# Autodesk Inventor assembly: Assembly
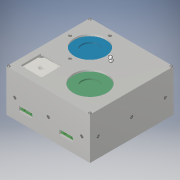
[picture p0: Inventor's stored thumbnail of the model, 180x180]
Saved by Autodesk Inventor 2018 (Build 220112000, 112)
## iProperties
Created: 2021-04-18
Part Number: Assembly
Document SubType Name: Assembly
Designer: Ramana Bharathi
Mass: 2974.86 g
Surface Area: 6185.71 cm^2
Volume: 1496.71 cm^3
Density: 1.9876 g/cm^3
Author: Ramana Bharathi
## Documents named in this file (17)
- E:\College\college material\4th sem\Machining and precision manufacturing\Assignments\task-1\Assembly.iam
- E:\College\college material\4th sem\Machining and precision manufacturing\Assignments\task-1\sensor3.ipt
- E:\College\college material\4th sem\Machining and precision manufacturing\Assignments\task-1\sensor1.ipt
- E:\College\college material\4th sem\Machining and precision manufacturing\Assignments\task-1\sensor2.ipt
- E:\College\college material\4th sem\Machining and precision manufacturing\Assignments\task-1\Housing_bottom.ipt
- E:\College\college material\4th sem\Machining and precision manufacturing\Assignments\task-1\spacer.ipt
- E:\College\college material\4th sem\Machining and precision manufacturing\Assignments\task-1\Board.ipt
- E:\College\college material\4th sem\Machining and precision manufacturing\Assignments\task-1\Housing_top.ipt
- E:\College\college material\4th sem\Machining and precision manufacturing\Assignments\task-1\Housing_lid.ipt
- E:\College\college material\4th sem\Machining and precision manufacturing\Assignments\task-1\sensor1_lock.ipt
- E:\College\college material\4th sem\Machining and precision manufacturing\Assignments\task-1\sensor3_lock.ipt
- E:\College\college material\4th sem\Machining and precision manufacturing\Assignments\task-1\sensor2_lock.ipt
- C:\Users\Ramana Bharathi\Documents\Inventor\Content Center Files\R2018\en-US\AS 1427(05)\AS 1427 - M3 x 8(5) II.ipt
- C:\Users\Ramana Bharathi\Documents\Inventor\Content Center Files\R2018\en-US\AS 1427(05)\AS 1427 - M4 x 6(5) II.ipt
- C:\Users\Ramana Bharathi\Documents\Inventor\Content Center Files\R2018\en-US\AS 1427(04)\AS 1427 - M3 x 16(5) I.ipt
- C:\Users\Ramana Bharathi\Documents\Inventor\Content Center Files\R2018\en-US\AS 1112 (2)\AS 1112 - M3  Type 5.ipt
- C:\Users\Ramana Bharathi\Documents\Inventor\Content Center Files\R2018\en-US\AS 1427(04)\AS 1427 - M4 x 8(5) I.ipt
## Components (63 placed, 16 different names)
1. sensor1:1 — Mate:2, Mate:3, Mate:5
2. sensor1:2 — Mate:4, Mate:5, Mate:7
3. sensor1:3 — Mate:6, Mate:7, Mate:8
4. sensor1:4 — Mate:1, Mate:8
5. sensor2:1 — Insert:16
6. sensor3:1 — Mate:46, Mate:47, Mate:48, Insert:12, Insert:13, Insert:14, Insert:15
7. Board:1 — Insert:17, Insert:18, Mate:63, Mate:65, Mate:67, Mate:69, Mate:71, Mate:73, Mate:77, Mate:79
8. Housing_bottom:1 — Insert:1, Insert:2, Insert:3, Insert:4, Insert:5, Insert:6, Insert:7, Insert:8, Insert:9, Flush:1, Flush:2, Mate:80, Mate:81, Mate:82, Mate:83, Mate:84, Mate:85, Mate:86, Mate:87, Mate:88, Mate:89, Mate:90, Mate:91, Mate:92
9. Housing_top:1 — Mate:40, Mate:41, Mate:42, Mate:43, Mate:44, Mate:45, Mate:53, Mate:54, Mate:55, Mate:60, Mate:61, Flush:1, Flush:2, Mate:80, Mate:93
10. Housing_lid:1 — Mate:9, Mate:10, Mate:11, Mate:12, Mate:36, Mate:37, Mate:38, Mate:39, Mate:60, Mate:61, Mate:93, Mate:94, Mate:95, Mate:96, Mate:97, Mate:98, Mate:99, Mate:100, Mate:101
11. spacer:1 — Insert:1, Insert:17, Mate:72
12. spacer:2 — Insert:2, Mate:68
13. spacer:3 — Insert:3, Mate:66
14. spacer:4 — Insert:4, Mate:76
15. spacer:5 — Insert:5
16. spacer:6 — Insert:6, Mate:64
17. spacer:7 — Insert:7, Mate:78
18. spacer:8 — Insert:8, Mate:70
19. spacer:9 — Insert:9, Insert:18, Mate:62
20. sensor1_lock:1 — Mate:1, Mate:2, Mate:3, Mate:4, Mate:6, Mate:9, Mate:10, Mate:11, Mate:12
21. AS 1427 H - Metric M4 x 8:11 — Mate:36
22. AS 1427 H - Metric M4 x 8:12 — Mate:37
23. AS 1427 H - Metric M4 x 8:13 — Mate:38
24. AS 1427 H - Metric M4 x 8:14 — Mate:39
25. sensor3_lock:1 — Mate:40, Mate:41, Mate:42, Mate:46, Mate:48, Insert:10, Insert:11
26. sensor3_lock:2 — Mate:43, Mate:44, Mate:45, Mate:47, Mate:49, Mate:50, Mate:51, Mate:52
27. sensor2_lock:1 — Mate:53, Mate:54, Insert:16, Mate:55, Mate:56, Mate:57, Mate:58, Mate:59
28. AS 1427 H - Metric M3 x 8:1 — Insert:10
29. AS 1427 H - Metric M3 x 8:2 — Insert:11
30. AS 1427 H - Metric M3 x 8:3 — Mate:49, Mate:50
31. AS 1427 H - Metric M3 x 8:4 — Mate:51, Mate:52
32. AS 1427 H - Metric M4 x 6:9 — Insert:12
33. AS 1427 H - Metric M4 x 6:10 — Insert:13
34. AS 1427 H - Metric M4 x 6:11 — Insert:14
35. AS 1427 H - Metric M4 x 6:12 — Insert:15
36. AS 1427 H - Metric M3 x 16:1 — Mate:56
37. AS 1427 H - Metric M3 x 16:2 — Mate:57
38. AS 1427 H - Metric M3 x 16:3 — Mate:58
39. AS 1427 H - Metric M3 x 16:4 — Mate:59
40. AS 1112 (2) - Metric M3  Type 5:1 — Mate:62, Mate:63
41. AS 1112 (2) - Metric M3  Type 5:2 — Mate:64, Mate:65
42. AS 1112 (2) - Metric M3  Type 5:3 — Mate:66, Mate:67
43. AS 1112 (2) - Metric M3  Type 5:4 — Mate:68, Mate:69
44. AS 1112 (2) - Metric M3  Type 5:5 — Mate:70, Mate:71
45. AS 1112 (2) - Metric M3  Type 5:6 — Mate:72, Mate:73
46. AS 1112 (2) - Metric M3  Type 5:8 — Mate:76, Mate:77
47. AS 1112 (2) - Metric M3  Type 5:9 — Mate:78, Mate:79
48. AS 1427 H - Metric M4 x 8:1 — Mate:81
49. AS 1427 H - Metric M4 x 8:2 — Mate:82
50. AS 1427 H - Metric M4 x 8:3 — Mate:83
51. AS 1427 H - Metric M4 x 8:4 — Mate:84
52. AS 1427 H - Metric M4 x 8:5 — Mate:85
53. AS 1427 H - Metric M4 x 8:6 — Mate:86
54. AS 1427 H - Metric M4 x 8:10 — Mate:87
55. AS 1427 H - Metric M4 x 8:15 — Mate:88
56. AS 1427 H - Metric M4 x 8:16 — Mate:89
57. AS 1427 H - Metric M4 x 8:7 — Mate:90
58. AS 1427 H - Metric M4 x 8:8 — Mate:91
59. AS 1427 H - Metric M4 x 8:9 — Mate:92
60. AS 1427 H - Metric M3 x 8:5 — Mate:94, Mate:95
61. AS 1427 H - Metric M3 x 8:6 — Mate:96, Mate:97
62. AS 1427 H - Metric M3 x 8:7 — Mate:98, Mate:99
63. AS 1427 H - Metric M3 x 8:8 — Mate:100, Mate:101
## Relationships (96: Mate 76, Insert 18, Flush 2)
- Insert:1: Housing_bottom:1 ↔ spacer:1
- Insert:2: Housing_bottom:1 ↔ spacer:2
- Insert:3: Housing_bottom:1 ↔ spacer:3
- Insert:4: Housing_bottom:1 ↔ spacer:4
- Insert:5: Housing_bottom:1 ↔ spacer:5
- Insert:6: Housing_bottom:1 ↔ spacer:6
- Insert:7: Housing_bottom:1 ↔ spacer:7
- Insert:8: Housing_bottom:1 ↔ spacer:8
- Insert:9: Housing_bottom:1 ↔ spacer:9
- Mate:1: sensor1:4 ↔ sensor1_lock:1
- Mate:2: sensor1:1 ↔ sensor1_lock:1
- Mate:3: sensor1:1 ↔ sensor1_lock:1
- Mate:4: sensor1:2 ↔ sensor1_lock:1
- Mate:5: sensor1:1 ↔ sensor1:2
- Mate:6: sensor1:3 ↔ sensor1_lock:1
- Mate:7: sensor1:2 ↔ sensor1:3
- Mate:8: sensor1:3 ↔ sensor1:4
- Mate:9: Housing_lid:1 ↔ sensor1_lock:1
- Mate:10: Housing_lid:1 ↔ sensor1_lock:1
- Mate:11: Housing_lid:1 ↔ sensor1_lock:1
- Mate:12: Housing_lid:1 ↔ sensor1_lock:1
- Mate:36: Housing_lid:1 ↔ AS 1427 H - Metric M4 x 8:11
- Mate:37: Housing_lid:1 ↔ AS 1427 H - Metric M4 x 8:12
- Mate:38: Housing_lid:1 ↔ AS 1427 H - Metric M4 x 8:13
- Mate:39: Housing_lid:1 ↔ AS 1427 H - Metric M4 x 8:14
- Mate:40: Housing_top:1 ↔ sensor3_lock:1
- Mate:41: Housing_top:1 ↔ sensor3_lock:1
- Mate:42: Housing_top:1 ↔ sensor3_lock:1
- Mate:43: Housing_top:1 ↔ sensor3_lock:2
- Mate:44: Housing_top:1 ↔ sensor3_lock:2
- Mate:45: Housing_top:1 ↔ sensor3_lock:2
- Mate:46: sensor3:1 ↔ sensor3_lock:1
- Mate:47: sensor3:1 ↔ sensor3_lock:2
- Mate:48: sensor3:1 ↔ sensor3_lock:1
- Insert:10: sensor3_lock:1 ↔ AS 1427 H - Metric M3 x 8:1
- Insert:11: sensor3_lock:1 ↔ AS 1427 H - Metric M3 x 8:2
- Mate:49: sensor3_lock:2 ↔ AS 1427 H - Metric M3 x 8:3
- Mate:50: sensor3_lock:2 ↔ AS 1427 H - Metric M3 x 8:3
- Mate:51: sensor3_lock:2 ↔ AS 1427 H - Metric M3 x 8:4
- Mate:52: sensor3_lock:2 ↔ AS 1427 H - Metric M3 x 8:4
- Insert:12: sensor3:1 ↔ AS 1427 H - Metric M4 x 6:9
- Insert:13: sensor3:1 ↔ AS 1427 H - Metric M4 x 6:10
- Insert:14: sensor3:1 ↔ AS 1427 H - Metric M4 x 6:11
- Insert:15: sensor3:1 ↔ AS 1427 H - Metric M4 x 6:12
- Mate:53: Housing_top:1 ↔ sensor2_lock:1
- Mate:54: Housing_top:1 ↔ sensor2_lock:1
- Insert:16: sensor2:1 ↔ sensor2_lock:1
- Mate:55: Housing_top:1 ↔ sensor2_lock:1
- Mate:56: sensor2_lock:1 ↔ AS 1427 H - Metric M3 x 16:1
- Mate:57: sensor2_lock:1 ↔ AS 1427 H - Metric M3 x 16:2
- Mate:58: sensor2_lock:1 ↔ AS 1427 H - Metric M3 x 16:3
- Mate:59: sensor2_lock:1 ↔ AS 1427 H - Metric M3 x 16:4
- Mate:60: Housing_top:1 ↔ Housing_lid:1
- Mate:61: Housing_top:1 ↔ Housing_lid:1
- Insert:17: Board:1 ↔ spacer:1
- Insert:18: Board:1 ↔ spacer:9
- Mate:62: spacer:9 ↔ AS 1112 (2) - Metric M3  Type 5:1
- Mate:63: Board:1 ↔ AS 1112 (2) - Metric M3  Type 5:1
- Mate:64: spacer:6 ↔ AS 1112 (2) - Metric M3  Type 5:2
- Mate:65: Board:1 ↔ AS 1112 (2) - Metric M3  Type 5:2
- Mate:66: spacer:3 ↔ AS 1112 (2) - Metric M3  Type 5:3
- Mate:67: Board:1 ↔ AS 1112 (2) - Metric M3  Type 5:3
- Mate:68: spacer:2 ↔ AS 1112 (2) - Metric M3  Type 5:4
- Mate:69: Board:1 ↔ AS 1112 (2) - Metric M3  Type 5:4
- Mate:70: spacer:8 ↔ AS 1112 (2) - Metric M3  Type 5:5
- Mate:71: Board:1 ↔ AS 1112 (2) - Metric M3  Type 5:5
- Mate:72: spacer:1 ↔ AS 1112 (2) - Metric M3  Type 5:6
- Mate:73: Board:1 ↔ AS 1112 (2) - Metric M3  Type 5:6
- Mate:76: spacer:4 ↔ AS 1112 (2) - Metric M3  Type 5:8
- Mate:77: Board:1 ↔ AS 1112 (2) - Metric M3  Type 5:8
- Mate:78: spacer:7 ↔ AS 1112 (2) - Metric M3  Type 5:9
- Mate:79: Board:1 ↔ AS 1112 (2) - Metric M3  Type 5:9
- Flush:1: Housing_bottom:1 ↔ Housing_top:1
- Flush:2: Housing_bottom:1 ↔ Housing_top:1
- Mate:80: Housing_bottom:1 ↔ Housing_top:1
- Mate:81: Housing_bottom:1 ↔ AS 1427 H - Metric M4 x 8:1
- Mate:82: Housing_bottom:1 ↔ AS 1427 H - Metric M4 x 8:2
- Mate:83: Housing_bottom:1 ↔ AS 1427 H - Metric M4 x 8:3
- Mate:84: Housing_bottom:1 ↔ AS 1427 H - Metric M4 x 8:4
- Mate:85: Housing_bottom:1 ↔ AS 1427 H - Metric M4 x 8:5
- Mate:86: Housing_bottom:1 ↔ AS 1427 H - Metric M4 x 8:6
- Mate:87: Housing_bottom:1 ↔ AS 1427 H - Metric M4 x 8:10
- Mate:88: Housing_bottom:1 ↔ AS 1427 H - Metric M4 x 8:15
- Mate:89: Housing_bottom:1 ↔ AS 1427 H - Metric M4 x 8:16
- Mate:90: Housing_bottom:1 ↔ AS 1427 H - Metric M4 x 8:7
- Mate:91: Housing_bottom:1 ↔ AS 1427 H - Metric M4 x 8:8
- Mate:92: Housing_bottom:1 ↔ AS 1427 H - Metric M4 x 8:9
- Mate:93: Housing_top:1 ↔ Housing_lid:1
- Mate:94: Housing_lid:1 ↔ AS 1427 H - Metric M3 x 8:5
- Mate:95: Housing_lid:1 ↔ AS 1427 H - Metric M3 x 8:5
- Mate:96: Housing_lid:1 ↔ AS 1427 H - Metric M3 x 8:6
- Mate:97: Housing_lid:1 ↔ AS 1427 H - Metric M3 x 8:6
- Mate:98: Housing_lid:1 ↔ AS 1427 H - Metric M3 x 8:7
- Mate:99: Housing_lid:1 ↔ AS 1427 H - Metric M3 x 8:7
- Mate:100: Housing_lid:1 ↔ AS 1427 H - Metric M3 x 8:8
- Mate:101: Housing_lid:1 ↔ AS 1427 H - Metric M3 x 8:8
